# Autodesk Inventor assembly: Joint Assembly
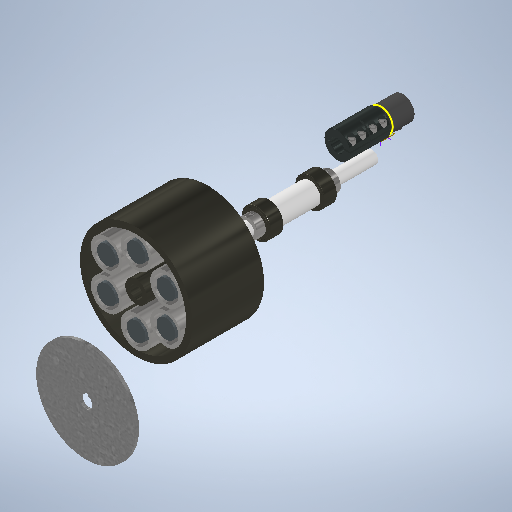
[picture p0: Inventor's stored thumbnail of the model, 512x512]
Saved by Autodesk Inventor 2025 (Build 290162000, 162)
## iProperties
Created: 2026-07-22
Part Number: Joint Assembly
Document SubType Name: Assembly
Designer: matot
Author: matot
## Documents named in this file (9)
- C:\Users\matot\OneDrive - Stellenbosch University\2026\MechatronicsProject478\Building the joint\Joint Assembly\Joint Assembly.iam
- C:\Users\matot\OneDrive - Stellenbosch University\2026\MechatronicsProject478\Building the joint\Joint Assembly\Brake disc.ipt
- C:\Users\matot\OneDrive - Stellenbosch University\2026\MechatronicsProject478\Building the joint\Joint Assembly\Electromagnet.iam
- C:\Users\matot\OneDrive - Stellenbosch University\2026\MechatronicsProject478\Building the joint\Joint Assembly\2058786.iam
- C:\Users\matot\OneDrive - Stellenbosch University\2026\MechatronicsProject478\Building the joint\Joint Assembly\mclx-20-20-f.iam
- C:\Users\matot\OneDrive - Stellenbosch University\2026\MechatronicsProject478\Building the joint\Joint Assembly\Reducer bushing.ipt
- C:\Users\matot\OneDrive - Stellenbosch University\2026\MechatronicsProject478\Building the joint\Joint Assembly\Optical Encoder.ipt
- C:\Users\matot\OneDrive - Stellenbosch University\2026\MechatronicsProject478\Building the joint\Joint Assembly\Rough draft shaft.ipt
- C:\Users\matot\OneDrive - Stellenbosch University\2026\MechatronicsProject478\Building the joint\Joint Assembly\8236976.ipt
## Components (10 placed, 8 different names)
1. Brake disc:1
2. Electromagnet:1 [sub-assembly]
3. 2058786:1 [sub-assembly] — Insert:5, Insert:7
4. 2058786:2 [sub-assembly] — Insert:6, Insert:8
5. mclx-20-20-f:1 [sub-assembly] — Mate:1, Insert:9
6. Reducer bushing:2 — Insert:2, Mate:1, Insert:9
7. Optical Encoder:1 — Insert:2
8. Rough draft shaft:1 — Insert:7, Insert:8
9. 8236976:1 — Insert:5
10. 8236976:2 — Insert:6
## Relationships (7: Insert 6, Mate 1)
- Insert:2: Reducer bushing:2 ↔ Optical Encoder:1
- Mate:1: mclx-20-20-f:1 ↔ Reducer bushing:2
- Insert:5: 2058786:1 ↔ 8236976:1
- Insert:6: 2058786:2 ↔ 8236976:2
- Insert:7: 2058786:1 ↔ Rough draft shaft:1
- Insert:8: 2058786:2 ↔ Rough draft shaft:1
- Insert:9: mclx-20-20-f:1 ↔ Reducer bushing:2
